# Autodesk Inventor assembly: main_assembly
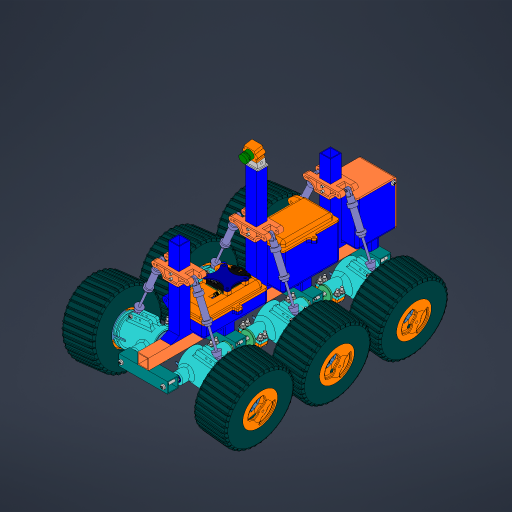
[picture p0: Inventor's stored thumbnail of the model, 512x512]
Saved by Autodesk Inventor 2024 (Build 280153000, 153)
## iProperties
Created: 2023-04-13
Part Number: main_assembly
Document SubType Name: Assembly
Designer: user
Mass: 4089.9 g
Surface Area: 11829.3 cm^2
Volume: 3903.66 cm^3
Density: 1.04771 g/cm^3
Author: user
## Documents named in this file (13)
- D:\Docs\Robot\3d\main_assembly.iam
- D:\Docs\Robot\3d\base\base_assembly.iam
- D:\Docs\Robot\3d\motor_assembly\default_motor_asembly.iam
- D:\Docs\Robot\3d\motor_assembly\holder_assembly.iam
- D:\Docs\Robot\3d\motor_assembly\rigt_motor_asembly.iam
- D:\Docs\Robot\3d\motor_assembly\left_motor_asembly.iam
- D:\Docs\Robot\3d\machine_body\front_box_asembly.iam
- D:\Docs\Robot\3d\machine_body\shock_absorber_holder_up.ipt
- D:\Docs\Robot\3d\machine_body\back_box_asembly.iam
- D:\Docs\Robot\3d\default_components\shock_absorber.ipt
- D:\Docs\Robot\3d\machine_body\tail_box_asembly.iam
- C:\Users\user\Documents\Inventor\Content Center Files\R2024\ru-RU\DIN 7985 (H)\DIN 7985 (H) - M4x30-H.ipt
- D:\Docs\Robot\3d\machine_body\cum_holders_mono\cum_holder_asembly.iam
## Components (28 placed, 12 different names)
1. base_assembly:1 [sub-assembly] — Совмещение:1, Совмещение:2, Совмещение:3, Совмещение:4, Вставка:1, Совмещение:5, Совмещение:6, Вставка:2, Вставка:3, Вставка:4, Вставка:5, Вставка:6, Совмещение:8, Совмещение:9, Заподлицо:1, Совмещение:10, Совмещение:11, Совмещение:12, Совмещение:13, Совмещение:14, Совмещение:15, Совмещение:16, Совмещение:18, Заподлицо:2, Совмещение:20, Заподлицо:3, Совмещение:21, Совмещение:26, Совмещение:27, Совмещение:28, Совмещение:33, Совмещение:34, Совмещение:35, Совмещение:36, Совмещение:37, Совмещение:38
2. default_motor_asembly:1 [sub-assembly] — Вставка:1, Совмещение:7, Совмещение:19
3. holder_assembly:1 [sub-assembly] — Совмещение:5, Совмещение:6, Совмещение:7
4. rigt_motor_asembly:1 [sub-assembly] — Вставка:2, Вставка:8
5. left_motor_asembly:1 [sub-assembly] — Вставка:3, Вставка:9
6. default_motor_asembly:2 [sub-assembly] — Вставка:4, Вставка:11
7. rigt_motor_asembly:2 [sub-assembly] — Вставка:5, Вставка:10
8. left_motor_asembly:2 [sub-assembly] — Вставка:6, Вставка:12
9. front_box_asembly:1 [sub-assembly] — Совмещение:8, Совмещение:9, Заподлицо:1
10. shock_absorber_holder_up:2 — Совмещение:10, Совмещение:11, Совмещение:22, Совмещение:28, Совмещение:29, Вставка:17, Вставка:18
11. shock_absorber_holder_up:3 — Совмещение:12, Совмещение:13, Вставка:7, Совмещение:25, Совмещение:27, Вставка:13, Вставка:14
12. shock_absorber_holder_up:4 — Совмещение:14, Совмещение:15, Совмещение:23, Совмещение:24, Совмещение:26, Вставка:15, Вставка:16
13. back_box_asembly:1 [sub-assembly] — Совмещение:16, Совмещение:18, Заподлицо:2
14. shock_absorber:1 — Вставка:7, Совмещение:19
15. tail_box_asembly:1 [sub-assembly] — Совмещение:20, Заподлицо:3, Совмещение:21
16. shock_absorber:2 — Совмещение:22, Вставка:8
17. shock_absorber:3 — Совмещение:23, Вставка:9
18. shock_absorber:4 — Совмещение:24, Вставка:10
19. shock_absorber:5 — Совмещение:25, Вставка:11
20. shock_absorber:6 — Вставка:12, Совмещение:29
21. holder_assembly:2 [sub-assembly] — Совмещение:33, Совмещение:34, Совмещение:35
22. DIN 7985 (H) M4x30-H:1 — Вставка:13
23. DIN 7985 (H) M4x30-H:2 — Вставка:14
24. DIN 7985 (H) M4x30-H:3 — Вставка:15
25. DIN 7985 (H) M4x30-H:4 — Вставка:16
26. DIN 7985 (H) M4x30-H:5 — Вставка:17
27. DIN 7985 (H) M4x30-H:6 — Вставка:18
28. cum_holder_asembly:1 [sub-assembly] — Совмещение:36, Совмещение:37, Совмещение:38
## Relationships (55: Mate 34, Insert 18, Flush 3)
- Совмещение:1 [Mate]: base_assembly:1
- Совмещение:2 [Mate]: base_assembly:1
- Совмещение:3 [Mate]: base_assembly:1
- Совмещение:4 [Mate]: base_assembly:1
- Вставка:1 [Insert] (11 mm): base_assembly:1 ↔ default_motor_asembly:1
- Совмещение:5 [Mate]: base_assembly:1 ↔ holder_assembly:1
- Совмещение:6 [Mate]: base_assembly:1 ↔ holder_assembly:1
- Совмещение:7 [Mate]: default_motor_asembly:1 ↔ holder_assembly:1
- Вставка:2 [Insert]: base_assembly:1 ↔ rigt_motor_asembly:1
- Вставка:3 [Insert]: base_assembly:1 ↔ left_motor_asembly:1
- Вставка:4 [Insert]: base_assembly:1 ↔ default_motor_asembly:2
- Вставка:5 [Insert]: base_assembly:1 ↔ rigt_motor_asembly:2
- Вставка:6 [Insert]: base_assembly:1 ↔ left_motor_asembly:2
- Совмещение:8 [Mate]: base_assembly:1 ↔ front_box_asembly:1
- Совмещение:9 [Mate]: base_assembly:1 ↔ front_box_asembly:1
- Заподлицо:1 [Flush]: base_assembly:1 ↔ front_box_asembly:1
- Совмещение:10 [Mate]: base_assembly:1 ↔ shock_absorber_holder_up:2
- Совмещение:11 [Mate]: base_assembly:1 ↔ shock_absorber_holder_up:2
- Совмещение:12 [Mate]: base_assembly:1 ↔ shock_absorber_holder_up:3
- Совмещение:13 [Mate]: base_assembly:1 ↔ shock_absorber_holder_up:3
- Совмещение:14 [Mate]: base_assembly:1 ↔ shock_absorber_holder_up:4
- Совмещение:15 [Mate]: base_assembly:1 ↔ shock_absorber_holder_up:4
- Совмещение:16 [Mate]: base_assembly:1 ↔ back_box_asembly:1
- Совмещение:18 [Mate]: base_assembly:1 ↔ back_box_asembly:1
- Заподлицо:2 [Flush]: base_assembly:1 ↔ back_box_asembly:1
- Вставка:7 [Insert]: shock_absorber_holder_up:3 ↔ shock_absorber:1
- Совмещение:19 [Mate]: default_motor_asembly:1 ↔ shock_absorber:1
- Совмещение:20 [Mate]: base_assembly:1 ↔ tail_box_asembly:1
- Заподлицо:3 [Flush]: base_assembly:1 ↔ tail_box_asembly:1
- Совмещение:21 [Mate]: base_assembly:1 ↔ tail_box_asembly:1
- Совмещение:22 [Mate]: shock_absorber_holder_up:2 ↔ shock_absorber:2
- Вставка:8 [Insert]: rigt_motor_asembly:1 ↔ shock_absorber:2
- Совмещение:23 [Mate]: shock_absorber_holder_up:4 ↔ shock_absorber:3
- Вставка:9 [Insert]: left_motor_asembly:1 ↔ shock_absorber:3
- Совмещение:24 [Mate]: shock_absorber_holder_up:4 ↔ shock_absorber:4
- Вставка:10 [Insert]: rigt_motor_asembly:2 ↔ shock_absorber:4
- Совмещение:25 [Mate]: shock_absorber_holder_up:3 ↔ shock_absorber:5
- Вставка:11 [Insert]: default_motor_asembly:2 ↔ shock_absorber:5
- Совмещение:26 [Mate] (40 mm): base_assembly:1 ↔ shock_absorber_holder_up:4
- Совмещение:27 [Mate] (90 mm): base_assembly:1 ↔ shock_absorber_holder_up:3
- Совмещение:28 [Mate] (40 mm): base_assembly:1 ↔ shock_absorber_holder_up:2
- Вставка:12 [Insert]: left_motor_asembly:2 ↔ shock_absorber:6
- Совмещение:29 [Mate]: shock_absorber_holder_up:2 ↔ shock_absorber:6
- Совмещение:33 [Mate]: base_assembly:1 ↔ holder_assembly:2
- Совмещение:34 [Mate]: base_assembly:1 ↔ holder_assembly:2
- Совмещение:35 [Mate]: base_assembly:1 ↔ holder_assembly:2
- Вставка:13 [Insert]: shock_absorber_holder_up:3 ↔ DIN 7985 (H) M4x30-H:1
- Вставка:14 [Insert]: shock_absorber_holder_up:3 ↔ DIN 7985 (H) M4x30-H:2
- Вставка:15 [Insert]: shock_absorber_holder_up:4 ↔ DIN 7985 (H) M4x30-H:3
- Вставка:16 [Insert]: shock_absorber_holder_up:4 ↔ DIN 7985 (H) M4x30-H:4
- Вставка:17 [Insert]: shock_absorber_holder_up:2 ↔ DIN 7985 (H) M4x30-H:5
- Вставка:18 [Insert]: shock_absorber_holder_up:2 ↔ DIN 7985 (H) M4x30-H:6
- Совмещение:36 [Mate]: base_assembly:1 ↔ cum_holder_asembly:1
- Совмещение:37 [Mate]: base_assembly:1 ↔ cum_holder_asembly:1
- Совмещение:38 [Mate]: base_assembly:1 ↔ cum_holder_asembly:1
